# Autodesk Inventor assembly: traction
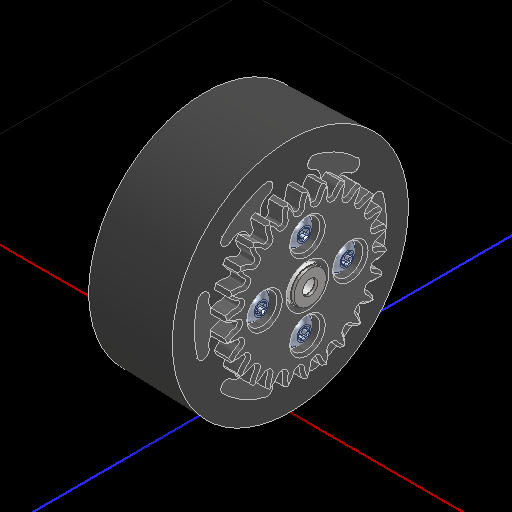
[picture p0: Inventor's stored thumbnail of the model, 512x512]
Saved by Autodesk Inventor 2025.2 (Build 292293000, 293)
## iProperties
Created: 2025-11-17
Part Number: traction
Document SubType Name: Assembly
Designer: cloudy
Author: cloudy
## Documents named in this file (10)
- C:\Users\cloudy\Documents\AURA_CAD\15\Drivetrain\Wheels\Traction\traction.iam
- C:\Users\cloudy\Documents\AURA_CAD\15\Drivetrain\Wheels\Traction\internal.ipt
- C:\Users\cloudy\Documents\AURA_CAD\15\Drivetrain\Wheels\Traction\tyre.ipt
- C:\Users\cloudy\Documents\AURA_CAD\!lib\Structure\Hardware\Nut Hex.ipt
- C:\Users\cloudy\Documents\AURA_CAD\!lib\Structure\Hardware\Screw Steel - Star\SScrew Star Threaded 1.000.ipt
- C:\Users\cloudy\Documents\AURA_CAD\!lib\Structure\Hardware\Screw Steel - Star.ipt
- C:\Users\cloudy\Documents\AURA_CAD\15\Drivetrain\Gears\26t.ipt
- C:\Users\cloudy\Documents\AURA_CAD\!lib\Motion\Insert Circle.ipt
- C:\Users\cloudy\Documents\AURA_CAD\!lib\Motion\Spacers\Washer Steel\SWasher .375 OD x .031250.ipt
- C:\Users\cloudy\Documents\AURA_CAD\!lib\Motion\Spacers\Washer Steel.ipt
## Components (16 placed, 7 different names)
1. internal:1 — Insert:1, Insert:2, Insert:3, Insert:4, Insert:5, Insert:10, Insert:12, Insert:13
2. tyre:1 — Insert:1
3. Nut Hex:1 — Insert:2
4. Nut Hex:2 — Insert:4
5. Nut Hex:3 — Insert:3
6. Nut Hex:4 — Insert:5
7. SScrew Star Threaded 1.000:1 — Insert:7
8. SScrew Star Threaded 1.000:2 — Insert:8
9. SScrew Star Threaded 1.000:3 — Insert:9
10. SScrew Star Threaded 1.000:4 — Insert:6
11. 26t:1 — Insert:6, Insert:7, Insert:8, Insert:9, Insert:11, Insert:13
12. Insert Circle:1 — Insert:10, Mate:1
13. Insert Circle:2 — Insert:11, Mate:1, Insert:14
14. Insert Circle:4 — Insert:12, Insert:15
15. SWasher .375 OD x .031250:1 — Insert:14
16. SWasher .375 OD x .031250:2 — Insert:15
## Relationships (16: Insert 15, Mate 1)
- Insert:1: internal:1 ↔ tyre:1
- Insert:2: internal:1 ↔ Nut Hex:1
- Insert:3: internal:1 ↔ Nut Hex:3
- Insert:4: internal:1 ↔ Nut Hex:2
- Insert:5: internal:1 ↔ Nut Hex:4
- Insert:6: SScrew Star Threaded 1.000:4 ↔ 26t:1
- Insert:7: SScrew Star Threaded 1.000:1 ↔ 26t:1
- Insert:8: SScrew Star Threaded 1.000:2 ↔ 26t:1
- Insert:9: SScrew Star Threaded 1.000:3 ↔ 26t:1
- Insert:10: internal:1 ↔ Insert Circle:1
- Insert:11: 26t:1 ↔ Insert Circle:2
- Insert:12: internal:1 ↔ Insert Circle:4
- Insert:13: internal:1 ↔ 26t:1
- Mate:1: Insert Circle:1 ↔ Insert Circle:2
- Insert:14: Insert Circle:2 ↔ SWasher .375 OD x .031250:1
- Insert:15: Insert Circle:4 ↔ SWasher .375 OD x .031250:2
